# Autodesk Inventor assembly: AS_GENERAL
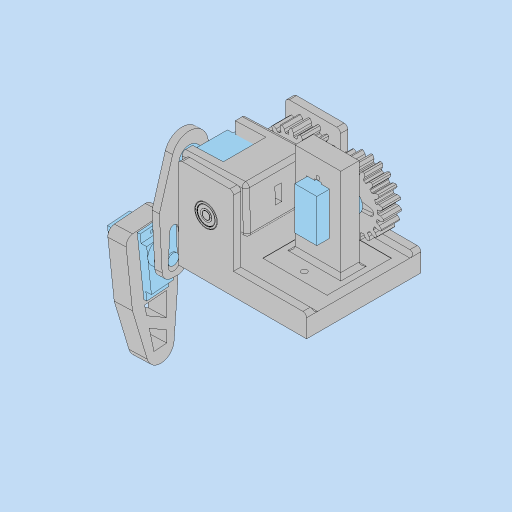
[picture p0: Inventor's stored thumbnail of the model, 512x512]
Saved by Autodesk Inventor 2024 (Build 280153000, 153)
## iProperties
Created: 2024-09-28
Part Number: AS_GENERAL
Document SubType Name: Assembly
Designer: MxMon
Author: MxMon
## Documents named in this file (16)
- C:\Users\MxMon\Documents\Inventor\CHEWIETRON\AS_GENERAL.iam
- C:\Users\MxMon\Documents\Inventor\CHEWIETRON\BASEPRINCIPAL_PATA_IZQ.ipt
- C:\Users\MxMon\Documents\Inventor\CHEWIETRON\bearing_604zz\bearing_604zz.ipt
- C:\Users\MxMon\Documents\Inventor\CHEWIETRON\BASEMOTOR_HOMBRO.ipt
- C:\Users\MxMon\Documents\Inventor\CHEWIETRON\Servo mockup\Servo mockup.ipt
- C:\Users\MxMon\Documents\Inventor\CHEWIETRON\Servo Motor hélice\Servo Motor hélice.ipt
- C:\Users\MxMon\Documents\Inventor\CHEWIETRON\PATA_SUP_IZQ.ipt
- C:\Users\MxMon\Documents\Inventor\CHEWIETRON\PARA_INF.ipt
- C:\Users\MxMon\Documents\Inventor\CHEWIETRON\BASEMOTOR_ENGRANE.ipt
- C:\Users\MxMon\Documents\Inventor\CHEWIETRON\CONECTOR_ENGRANE_HOMBRO.ipt
- C:\Users\MxMon\Documents\Inventor\CHEWIETRON\ENGRANE_HOMBRO.ipt
- C:\Users\MxMon\Documents\Inventor\CHEWIETRON\HELICE_CRUZ.ipt
- C:\Users\MxMon\Documents\Inventor\CHEWIETRON\ENGRANE_HELICE.ipt
- C:\Users\MxMon\Documents\Inventor\CHEWIETRON\EJE_TORNILLO.ipt
- C:\Users\MxMon\Documents\Inventor\CHEWIETRON\TUERCA.ipt
- C:\Users\MxMon\Documents\Inventor\CHEWIETRON\ESPACIADOR.ipt
## Components (19 placed, 15 different names)
1. BASEPRINCIPAL_PATA_IZQ:1 — Mate:1, Mate:2, Mate:3, Mate:4, Mate:23, Mate:25, Mate:46
2. bearing_604zz:1 — Mate:1, Mate:2, Mate:5, Mate:39, Mate:40
3. bearing_604zz:2 — Mate:3, Mate:4, Mate:44
4. BASEMOTOR_HOMBRO:1 — Mate:5, Mate:6, Mate:7, Mate:8, Mate:26, Mate:27, Mate:28, Mate:42
5. Servo mockup:1 — Mate:6, Mate:7, Mate:8, Mate:9, Mate:10
6. Servo Motor hélice:1 — Mate:9, Mate:10, Mate:11, Mate:12, Mate:13
7. PATA_SUP_IZQ:1 — Mate:11, Mate:12, Mate:13, Mate:47, Mate:48, Mate:49, Mate:50
8. Servo mockup:2 — Mate:20, Mate:21, Mate:22
9. Servo Motor hélice:2 — Mate:47, Mate:48, Mate:49, Mate:50
10. PARA_INF:1 — Mate:20, Mate:21, Mate:22
11. BASEMOTOR_ENGRANE:1 — Mate:23, Mate:25, Mate:36, Mate:37, Mate:38, Mate:46
12. CONECTOR_ENGRANE_HOMBRO:1 — Mate:26, Mate:27, Mate:28, Mate:29, Mate:30, Mate:31
13. ENGRANE_HOMBRO:1 — Mate:29, Mate:30, Mate:31
14. Servo mockup:3 — Mate:32, Mate:33, Mate:36, Mate:37, Mate:38
15. HELICE_CRUZ:1 — Mate:32, Mate:33, Mate:34, Mate:35
16. ENGRANE_HELICE:1 — Mate:34, Mate:35
17. EJE_TORNILLO:1 — Mate:39, Mate:40, Mate:41, Mate:43
18. TUERCA:1 — Mate:41, Mate:42, Mate:45
19. ESPACIADOR:1 — Mate:43, Mate:44, Mate:45
## Relationships (45: Mate 45)
- Mate:1: BASEPRINCIPAL_PATA_IZQ:1 ↔ bearing_604zz:1
- Mate:2: BASEPRINCIPAL_PATA_IZQ:1 ↔ bearing_604zz:1
- Mate:3: BASEPRINCIPAL_PATA_IZQ:1 ↔ bearing_604zz:2
- Mate:4: BASEPRINCIPAL_PATA_IZQ:1 ↔ bearing_604zz:2
- Mate:5: bearing_604zz:1 ↔ BASEMOTOR_HOMBRO:1
- Mate:6: BASEMOTOR_HOMBRO:1 ↔ Servo mockup:1
- Mate:7: BASEMOTOR_HOMBRO:1 ↔ Servo mockup:1
- Mate:8: BASEMOTOR_HOMBRO:1 ↔ Servo mockup:1
- Mate:9: Servo mockup:1 ↔ Servo Motor hélice:1
- Mate:10: Servo mockup:1 ↔ Servo Motor hélice:1
- Mate:11: Servo Motor hélice:1 ↔ PATA_SUP_IZQ:1
- Mate:12: Servo Motor hélice:1 ↔ PATA_SUP_IZQ:1
- Mate:13: Servo Motor hélice:1 ↔ PATA_SUP_IZQ:1
- [Mate]: Servo mockup:2 ↔ Servo Motor hélice:2
- [Mate]: Servo mockup:2 ↔ Servo Motor hélice:2
- Mate:20: Servo mockup:2 ↔ PARA_INF:1
- Mate:21: Servo mockup:2 ↔ PARA_INF:1
- Mate:22: Servo mockup:2 ↔ PARA_INF:1
- Mate:23: BASEPRINCIPAL_PATA_IZQ:1 ↔ BASEMOTOR_ENGRANE:1
- Mate:25: BASEPRINCIPAL_PATA_IZQ:1 ↔ BASEMOTOR_ENGRANE:1
- Mate:26: BASEMOTOR_HOMBRO:1 ↔ CONECTOR_ENGRANE_HOMBRO:1
- Mate:27: BASEMOTOR_HOMBRO:1 ↔ CONECTOR_ENGRANE_HOMBRO:1
- Mate:28: BASEMOTOR_HOMBRO:1 ↔ CONECTOR_ENGRANE_HOMBRO:1
- Mate:29: CONECTOR_ENGRANE_HOMBRO:1 ↔ ENGRANE_HOMBRO:1
- Mate:30: CONECTOR_ENGRANE_HOMBRO:1 ↔ ENGRANE_HOMBRO:1
- Mate:31: CONECTOR_ENGRANE_HOMBRO:1 ↔ ENGRANE_HOMBRO:1
- Mate:32: Servo mockup:3 ↔ HELICE_CRUZ:1
- Mate:33: Servo mockup:3 ↔ HELICE_CRUZ:1
- Mate:34: HELICE_CRUZ:1 ↔ ENGRANE_HELICE:1
- Mate:35: HELICE_CRUZ:1 ↔ ENGRANE_HELICE:1
- Mate:36: BASEMOTOR_ENGRANE:1 ↔ Servo mockup:3
- Mate:37: BASEMOTOR_ENGRANE:1 ↔ Servo mockup:3
- Mate:38: BASEMOTOR_ENGRANE:1 ↔ Servo mockup:3
- Mate:39: bearing_604zz:1 ↔ EJE_TORNILLO:1
- Mate:40: bearing_604zz:1 ↔ EJE_TORNILLO:1
- Mate:41: EJE_TORNILLO:1 ↔ TUERCA:1
- Mate:42: BASEMOTOR_HOMBRO:1 ↔ TUERCA:1
- Mate:43: EJE_TORNILLO:1 ↔ ESPACIADOR:1
- Mate:44: bearing_604zz:2 ↔ ESPACIADOR:1
- Mate:45: TUERCA:1 ↔ ESPACIADOR:1
- Mate:46: BASEPRINCIPAL_PATA_IZQ:1 ↔ BASEMOTOR_ENGRANE:1
- Mate:47: PATA_SUP_IZQ:1 ↔ Servo Motor hélice:2
- Mate:48: PATA_SUP_IZQ:1 ↔ Servo Motor hélice:2
- Mate:49: PATA_SUP_IZQ:1 ↔ Servo Motor hélice:2
- Mate:50: PATA_SUP_IZQ:1 ↔ Servo Motor hélice:2
## Named parameters: d16_d8 = 0 mm, d17_d9 = 0 mm
